# Autodesk Inventor assembly: Hexapod v0.1
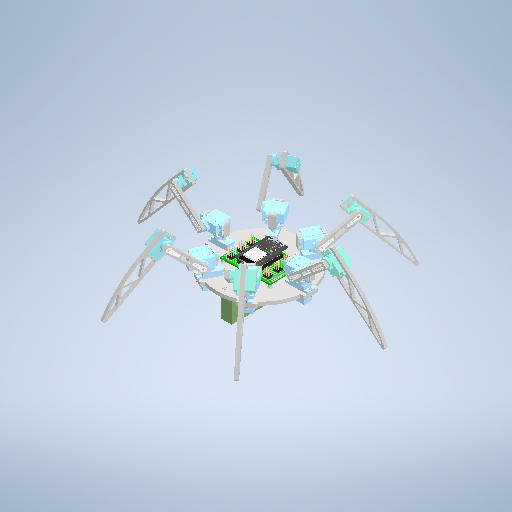
[picture p0: Inventor's stored thumbnail of the model, 512x512]
Saved by Autodesk Inventor 2025 (Build 290162000, 162)
## iProperties
Created: 2024-06-04
Part Number: Hexapod v0.1
Document SubType Name: Assembly
Designer: sgols
Author: sgols
## Documents named in this file (8)
- C:\git\hexapod\mechanics\Hexapod v0.1.iam
- C:\git\hexapod\mechanics\Base Plate v0.1.ipt
- C:\git\hexapod\mechanics\Leg Left v0.1.iam
- C:\git\hexapod\mechanics\Leg Right v0.1.iam
- C:\git\hexapod\mechanics\Electronics Control Board v0.1.iam
- C:\Users\sgols\Documents\Inventor\Content Center Files\R2025\en-US\DIN 7985 (H)\DIN 7985 (H) - M2x10-H.ipt
- C:\Users\sgols\Documents\Inventor\Content Center Files\R2025\en-US\DIN 934\DIN 934 - M2 x 0,4.ipt
- C:\git\hexapod\mechanics\LiFe Battery Blockout v0.1.ipt
## Components (33 placed, 7 different names)
1. Base Plate v0.1:1 — Mate:1, Mate:7, Mate:9, Mate:11, Mate:12, Mate:13, Mate:16, Mate:19, Insert:13, Insert:14, Mate:23, Mate:24, Mate:25, Mate:26, Mate:27, Mate:28, Angle:1, Angle:2, Angle:3, Angle:4, Angle:5, Angle:6, Insert:28, Insert:33, Insert:34, Insert:35, Insert:36, Insert:37, Insert:38, Insert:39, Insert:40, Insert:41, Insert:42, Insert:43, Mate:29
2. Electronics Control Board v0.1:1 [sub-assembly] — Insert:13, Insert:14
3. DIN 7985 (H) M2x10-H:1 — Insert:16
4. DIN 7985 (H) M2x10-H:2 — Insert:17
5. DIN 7985 (H) M2x10-H:3 — Insert:18
6. DIN 7985 (H) M2x10-H:4 — Insert:19
7. DIN 7985 (H) M2x10-H:5 — Insert:20
8. DIN 7985 (H) M2x10-H:6 — Insert:21
9. DIN 7985 (H) M2x10-H:7 — Insert:22
10. DIN 7985 (H) M2x10-H:8 — Insert:23
11. DIN 7985 (H) M2x10-H:9 — Insert:24
12. DIN 7985 (H) M2x10-H:10 — Insert:25
13. DIN 7985 (H) M2x10-H:11 — Insert:26
14. DIN 7985 (H) M2x10-H:12 — Insert:27
15. DIN 934 - replaced by DIN EN 24032/28673/28674 M2:1 — Insert:28
16. DIN 934 - replaced by DIN EN 24032/28673/28674 M2:6 — Insert:33
17. DIN 934 - replaced by DIN EN 24032/28673/28674 M2:7 — Insert:34
18. DIN 934 - replaced by DIN EN 24032/28673/28674 M2:8 — Insert:35
19. DIN 934 - replaced by DIN EN 24032/28673/28674 M2:9 — Insert:36
20. DIN 934 - replaced by DIN EN 24032/28673/28674 M2:10 — Insert:37
21. DIN 934 - replaced by DIN EN 24032/28673/28674 M2:11 — Insert:38
22. DIN 934 - replaced by DIN EN 24032/28673/28674 M2:12 — Insert:39
23. DIN 934 - replaced by DIN EN 24032/28673/28674 M2:13 — Insert:40
24. DIN 934 - replaced by DIN EN 24032/28673/28674 M2:14 — Insert:41
25. DIN 934 - replaced by DIN EN 24032/28673/28674 M2:15 — Insert:42
26. DIN 934 - replaced by DIN EN 24032/28673/28674 M2:16 — Insert:43
27. LiFe Battery Blockout v0.1:1 — Mate:29
28. Leg Left v0.1:1 [sub-assembly] — Mate:9, Mate:23, Angle:1, Insert:20, Insert:21
29. Leg Left v0.1:2 [sub-assembly] — Mate:1, Mate:24, Angle:2, Insert:18, Insert:19
30. Leg Left v0.1:3 [sub-assembly] — Mate:7, Mate:25, Angle:3, Insert:16, Insert:17
31. Leg Right v0.1:1 [sub-assembly] — Mate:13, Mate:26, Angle:4, Insert:22, Insert:23
32. Leg Right v0.1:2 [sub-assembly] — Mate:16, Mate:27, Angle:5, Insert:24, Insert:25
33. Leg Right v0.1:3 [sub-assembly] — Mate:19, Mate:28, Angle:6, Insert:26, Insert:27
## Relationships (47: Insert 26, Mate 15, Angle 6)
- Mate:1: Base Plate v0.1:1 ↔ Leg Left v0.1:2
- Mate:7: Base Plate v0.1:1 ↔ Leg Left v0.1:3
- Mate:9: Base Plate v0.1:1 ↔ Leg Left v0.1:1
- Mate:11: Base Plate v0.1:1
- Mate:12: Base Plate v0.1:1
- Mate:13: Base Plate v0.1:1 ↔ Leg Right v0.1:1
- Mate:16: Base Plate v0.1:1 ↔ Leg Right v0.1:2
- Mate:19: Base Plate v0.1:1 ↔ Leg Right v0.1:3
- Insert:13: Base Plate v0.1:1 ↔ Electronics Control Board v0.1:1
- Insert:14: Base Plate v0.1:1 ↔ Electronics Control Board v0.1:1
- Mate:23: Base Plate v0.1:1 ↔ Leg Left v0.1:1
- Mate:24: Base Plate v0.1:1 ↔ Leg Left v0.1:2
- Mate:25: Base Plate v0.1:1 ↔ Leg Left v0.1:3
- Mate:26: Base Plate v0.1:1 ↔ Leg Right v0.1:1
- Mate:27: Base Plate v0.1:1 ↔ Leg Right v0.1:2
- Mate:28: Base Plate v0.1:1 ↔ Leg Right v0.1:3
- Angle:1 (180 deg): Base Plate v0.1:1 ↔ Leg Left v0.1:1
- Angle:2 (180 deg): Base Plate v0.1:1 ↔ Leg Left v0.1:2
- Angle:3 (180 deg): Base Plate v0.1:1 ↔ Leg Left v0.1:3
- Angle:4 (180 deg): Base Plate v0.1:1 ↔ Leg Right v0.1:1
- Angle:5 (180 deg): Base Plate v0.1:1 ↔ Leg Right v0.1:2
- Angle:6 (180 deg): Base Plate v0.1:1 ↔ Leg Right v0.1:3
- Insert:16: DIN 7985 (H) M2x10-H:1 ↔ Leg Left v0.1:3
- Insert:17: DIN 7985 (H) M2x10-H:2 ↔ Leg Left v0.1:3
- Insert:18: DIN 7985 (H) M2x10-H:3 ↔ Leg Left v0.1:2
- Insert:19: DIN 7985 (H) M2x10-H:4 ↔ Leg Left v0.1:2
- Insert:20: DIN 7985 (H) M2x10-H:5 ↔ Leg Left v0.1:1
- Insert:21: DIN 7985 (H) M2x10-H:6 ↔ Leg Left v0.1:1
- Insert:22: DIN 7985 (H) M2x10-H:7 ↔ Leg Right v0.1:1
- Insert:23: DIN 7985 (H) M2x10-H:8 ↔ Leg Right v0.1:1
- Insert:24: DIN 7985 (H) M2x10-H:9 ↔ Leg Right v0.1:2
- Insert:25: DIN 7985 (H) M2x10-H:10 ↔ Leg Right v0.1:2
- Insert:26: DIN 7985 (H) M2x10-H:11 ↔ Leg Right v0.1:3
- Insert:27: DIN 7985 (H) M2x10-H:12 ↔ Leg Right v0.1:3
- Insert:28: Base Plate v0.1:1 ↔ DIN 934 - replaced by DIN EN 24032/28673/28674 M2:1
- Insert:33: Base Plate v0.1:1 ↔ DIN 934 - replaced by DIN EN 24032/28673/28674 M2:6
- Insert:34: Base Plate v0.1:1 ↔ DIN 934 - replaced by DIN EN 24032/28673/28674 M2:7
- Insert:35: Base Plate v0.1:1 ↔ DIN 934 - replaced by DIN EN 24032/28673/28674 M2:8
- Insert:36: Base Plate v0.1:1 ↔ DIN 934 - replaced by DIN EN 24032/28673/28674 M2:9
- Insert:37: Base Plate v0.1:1 ↔ DIN 934 - replaced by DIN EN 24032/28673/28674 M2:10
- Insert:38: Base Plate v0.1:1 ↔ DIN 934 - replaced by DIN EN 24032/28673/28674 M2:11
- Insert:39: Base Plate v0.1:1 ↔ DIN 934 - replaced by DIN EN 24032/28673/28674 M2:12
- Insert:40: Base Plate v0.1:1 ↔ DIN 934 - replaced by DIN EN 24032/28673/28674 M2:13
- Insert:41: Base Plate v0.1:1 ↔ DIN 934 - replaced by DIN EN 24032/28673/28674 M2:14
- Insert:42: Base Plate v0.1:1 ↔ DIN 934 - replaced by DIN EN 24032/28673/28674 M2:15
- Insert:43: Base Plate v0.1:1 ↔ DIN 934 - replaced by DIN EN 24032/28673/28674 M2:16
- Mate:29: Base Plate v0.1:1 ↔ LiFe Battery Blockout v0.1:1
